# Autodesk Inventor assembly: canaletaIzquierda
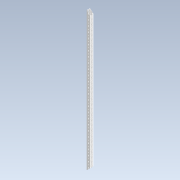
[picture p0: Inventor's stored thumbnail of the model, 180x180]
Saved by Autodesk Inventor 2021 (Build 250183000, 183)
## iProperties
Created: 2021-07-13
Part Number: canaletaIzquierda
Document SubType Name: Assembly
Designer: Andrés Holguín
Author: Andrés Holguín
## Documents named in this file (2)
- C:\Users\andre\Documents\GitHub\Dis.-Mecatronico-E6\inventor proyecto\Tablero\Canaletas\canaletaIzquierda.iam
- C:\Users\andre\Documents\GitHub\Dis.-Mecatronico-E6\inventor proyecto\Tablero\Canaletas\7308-1.iam
## Components (13 placed, 1 different names)
1. 7308-1:3 [sub-assembly] — Rigid:3, Mate:2, Angle:2
2. 7308-1:4 [sub-assembly] — Rigid:3, Rigid:4
3. 7308-1:5 [sub-assembly] — Mate:1, Rigid:7, Rigid:8
4. 7308-1:6 [sub-assembly] — Rigid:4, Rigid:5
5. 7308-1:7 [sub-assembly] — Rigid:5, Rigid:9
6. 7308-1:8 [sub-assembly] — Rigid:6, Rigid:7
7. 7308-1:9 [sub-assembly] — Rigid:8, Mate:3, Angle:3, Rigid:13
8. 7308-1:10 [sub-assembly] — Rigid:6, Rigid:10
9. 7308-1:11 [sub-assembly] — Rigid:9, Rigid:10
10. 7308-1:12 [sub-assembly] — Rigid:12, Rigid:13
11. 7308-1:13 [sub-assembly] — Rigid:11, Rigid:14
12. 7308-1:14 [sub-assembly] — Rigid:11, Rigid:12
13. 7308-1:15 [sub-assembly] — Rigid:14, Mate:4, Angle:4
## Relationships (19: WeldJoint 12, Mate 4, Angle 3)
- Rigid:3 [WeldJoint]: 7308-1:3 ↔ 7308-1:4
- Mate:1: 7308-1:5
- Mate:2: 7308-1:3
- Angle:2 (45 deg): 7308-1:3
- Rigid:4 [WeldJoint]: 7308-1:4 ↔ 7308-1:6
- Rigid:5 [WeldJoint]: 7308-1:6 ↔ 7308-1:7
- Rigid:6 [WeldJoint]: 7308-1:8 ↔ 7308-1:10
- Rigid:7 [WeldJoint]: 7308-1:5 ↔ 7308-1:8
- Rigid:8 [WeldJoint]: 7308-1:5 ↔ 7308-1:9
- Mate:3: 7308-1:9
- Angle:3 (45 deg): 7308-1:9
- Rigid:9 [WeldJoint]: 7308-1:7 ↔ 7308-1:11
- Rigid:10 [WeldJoint]: 7308-1:10 ↔ 7308-1:11
- Rigid:11 [WeldJoint]: 7308-1:13 ↔ 7308-1:14
- Rigid:12 [WeldJoint]: 7308-1:12 ↔ 7308-1:14
- Rigid:13 [WeldJoint]: 7308-1:9 ↔ 7308-1:12
- Rigid:14 [WeldJoint]: 7308-1:13 ↔ 7308-1:15
- Mate:4: 7308-1:15
- Angle:4 (45 deg): 7308-1:15
